# Autodesk Inventor assembly: Drill
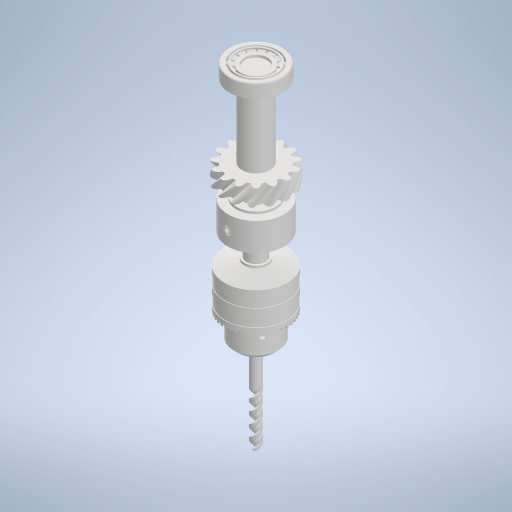
[picture p0: Inventor's stored thumbnail of the model, 512x512]
Saved by Autodesk Inventor 2024.2 (Build 282272000, 272)
## iProperties
Created: 2021-09-13
Part Number: Drill
Description: STEP AP203
Document SubType Name: Assembly
Designer: 062210026
Sending System: SolidWorks 2018
Preprocessor: SwSTEP 2.0
Title: multi-spindle.STEP
Author: Moghimi
Revision Number: ANY
## Documents named in this file (7)
- Z:\ProjInt3\Ferramenta\Drill.iam
- Z:\ProjInt3\Maquina\maquina\15_Varsay_lan.ipt
- Z:\ProjInt3\Maquina\maquina\SKF_30204.iam
- Z:\ProjInt3\Maquina\maquina\6-AX.ipt
- Z:\ProjInt3\Maquina\maquina\helical gear_3_am2_Metric - RH Helical gear 2.5M 15T 45HA 20PA 15FW ---15N75H50L25.0R1.ipt
- Z:\ProjInt3\Maquina\maquina\spring pin slotted_ai_SPS 0.25x1.25.ipt
- Z:\ProjInt3\Ferramenta\Escalonada1.ipt
## Components (6 placed, 6 different names)
1. Escalonada1:1 — Mate:1
2. SKF_30204:7 [sub-assembly]
3. helical gear_3_am2_Metric - RH Helical gear 2.5M 15T 45HA 20PA 15FW ---15N75H50L25.0R1:7
4. 6-AX:7
5. spring pin slotted_ai_SPS 0.25x1.25:7
6. 15_Varsay_lan:8 — Mate:1
## Relationships (1: Mate 1)
- Mate:1: Escalonada1:1 ↔ 15_Varsay_lan:8
